# Autodesk Inventor assembly: Lumipositor2-Assy
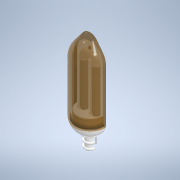
[picture p0: Inventor's stored thumbnail of the model, 180x180]
Saved by Autodesk Inventor 2022 (Build 260153000, 153)
## iProperties
Created: 2021-10-27
Part Number: Lumipositor2-Assy
Document SubType Name: Assembly
Designer: incep
Author: incep
## Documents named in this file (5)
- C:\Users\incep\Desktop\3D Printer Stuff\TheLightWithinYou\Lumipositor2-Assy.iam
- C:\Users\incep\Desktop\3D Printer Stuff\TheLightWithinYou\Lumipositor2-Bottom-V1.ipt
- C:\Users\incep\Desktop\3D Printer Stuff\TheLightWithinYou\Lumipositor2-Top-V1.ipt
- C:\Users\incep\Desktop\3D Printer Stuff\TheLightWithinYou\R-21-O-ring.ipt
- C:\Users\incep\Desktop\3D Printer Stuff\TheLightWithinYou\Flashbulb-DU8902.ipt
## Components (4 placed, 4 different names)
1. Lumipositor2-Bottom-V1:1 — Mate:1, Mate:2, Mate:3, Mate:4, Mate:5, Symmetry:1, Mate:8, Mate:9
2. Lumipositor2-Top-V1:1 — Mate:1, Mate:3, Symmetry:1
3. R-21-O-ring:1 — Mate:2, Angle:1, Mate:6
4. Flashbulb-DU8902:1 — Mate:8, Mate:9
## Relationships (11: Mate 9, Angle 1, Symmetry 1)
- Mate:1: Lumipositor2-Bottom-V1:1 ↔ Lumipositor2-Top-V1:1
- Mate:2: Lumipositor2-Bottom-V1:1 ↔ R-21-O-ring:1
- Mate:3: Lumipositor2-Bottom-V1:1 ↔ Lumipositor2-Top-V1:1
- Mate:4: Lumipositor2-Bottom-V1:1
- Mate:5: Lumipositor2-Bottom-V1:1
- Angle:1 (0 deg): R-21-O-ring:1
- Mate:6: R-21-O-ring:1
- Symmetry:1: Lumipositor2-Bottom-V1:1 ↔ Lumipositor2-Top-V1:1
- Mate:7
- Mate:8: Lumipositor2-Bottom-V1:1 ↔ Flashbulb-DU8902:1
- Mate:9: Lumipositor2-Bottom-V1:1 ↔ Flashbulb-DU8902:1
